# Autodesk Inventor assembly: AXb1
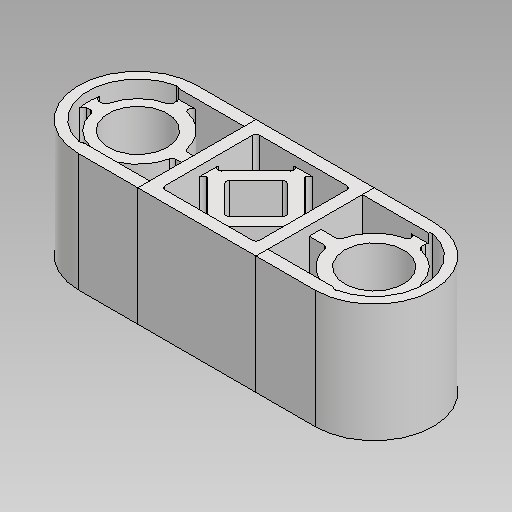
[picture p0: Inventor's stored thumbnail of the model, 512x512]
Saved by Autodesk Inventor 2020 (Build 240168000, 168)
## iProperties
Created: 2019-05-06
Part Number: AXb1
Document SubType Name: Assembly
Designer: Varga Daniel
Author: Varga Daniel
## Documents named in this file (3)
- C:\!_Dani\!_cloud\OneDrive\!_munka\Revolution\StructuralParts\Beams\Axle Beams\AXb1.iam
- C:\!_Dani\!_cloud\OneDrive\!_munka\Revolution\StructuralParts\Beams\Axle Beams\Axle beam base.ipt
- C:\!_Dani\!_cloud\OneDrive\!_munka\Revolution\StructuralParts\Beams\beam_single_end_part.ipt
## Components (3 placed, 2 different names)
1. Axle beam base:1 — Mate:1, Mate:2, Flush:1, Mate:3, Mate:4, Flush:2, Flush:4, Flush:7, Flush:9
2. beam_single_end_part:1 — Mate:4, Flush:2, Flush:9
3. beam_single_end_part:4 — Mate:3, Flush:4, Flush:7
## Relationships (9: Flush 5, Mate 4)
- Mate:1: Axle beam base:1
- Mate:2: Axle beam base:1
- Flush:1: Axle beam base:1
- Mate:3: Axle beam base:1 ↔ beam_single_end_part:4
- Mate:4: Axle beam base:1 ↔ beam_single_end_part:1
- Flush:2: Axle beam base:1 ↔ beam_single_end_part:1
- Flush:4: Axle beam base:1 ↔ beam_single_end_part:4
- Flush:7: Axle beam base:1 ↔ beam_single_end_part:4
- Flush:9: Axle beam base:1 ↔ beam_single_end_part:1
